# Autodesk Inventor assembly: C-SHA10_MIR_MIR_MIR1
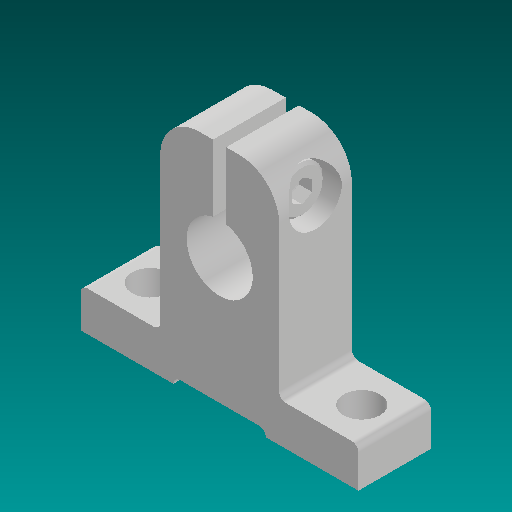
[picture p0: Inventor's stored thumbnail of the model, 512x512]
Saved by Autodesk Inventor 2020 (Build 240168000, 168)
## iProperties
Category: PARTsolutions
Company: MISUMI
Created: 2022-11-04
Part Number: C-SHA10_MIR_MIR_MIR1
Catalog Web Link: www.cadenas.de
Description: C-SHA-Economy Shaft Supports - T-Shaped/Slit
Vendor: MISUMI
Document SubType Name: Assembly
Designer: kanazawakotaro
Manufacturer: MISUMI
Mass: 6.70187 g
Surface Area: 40.5742 cm^2
Volume: 6.70187 cm^3
Density: 1 g/cm^3
Title: C-SHA10
Author: Cadenas PARTsolutions
Comments: Economy Shaft Supports - T-Shaped/Slit
PSOL_IDENT_0: {$CADENAS_DATA/23d-libs/misumi/metric/02_shaft_supports/c_sha_asmtab.prj},167 {VTYP=3D},{STYP=ASSTAB
PSOL_IDENT_1: },{NB=C-SHA10},{LINA=C-SHA10},{NN=C-SHA},{DATE=04.10.2022 06:54:20},{GEOMDATE=23.04.2021 02:50:35},{
PSOL_IDENT_2: VERSION=},{LINEID=10},{WBVAR=},{WBNUMERIC=}  {NB=C-SHA10},{LINA=C-SHA10},{KT=DUMMY},{PN=C-SHA10},{TY
PSOL_IDENT_3: PE=C-SHA},{D=10},{H=20},{H1=35},{T=11},{L1=32},{DD=5.5},{E=9.5},{S=6},{R=6},{L=42},{B=14},{W=18},{M=
PSOL_IDENT_4: M4},{R2=1},{W2=2.0},{M3D=4},{M3D2=6.0},{M3D3=8},{M3D4=4.3},{LB=10},{PPATH=c_sha/c_sha_asmtpl.prj}
NB: C-SHA10
NN: C-SHA
NT: Economy Shaft Supports - T-Shaped/Slit
NBSYN: $PN.
LINA: C-SHA10
CATALOG: Misumi
PN: C-SHA10
D: 10
H: 20
H1: 35
T: 11
L1: 32
DD: 5.5
E: 9.5
S: 6
R: 6
L: 42
B: 14
W: 18
M: M4
SUPPLIER: MISUMI
ARTICLENO: C-SHA10
BOMINFO: C-SHA10
CREATOR: CADENAS GmbH
## Documents named in this file (3)
- C:\Users\金澤航太郎\Documents\Inventor\kamuy2\Parts\C-SHA10_Autodesk_Inventor_2020_20221104\AIS2020\C-SHA10_MIR_MIR_MIR1.iam
- C:\Users\金澤航太郎\Documents\Inventor\kamuy2\Parts\C-SHA10_Autodesk_Inventor_2020_20221104\AIS2020\C-SHA10_b_MIR_MIR_MIR1.ipt
- C:\Users\金澤航太郎\Documents\Inventor\kamuy2\Parts\C-SHA10_Autodesk_Inventor_2020_20221104\AIS2020\BOLT4-10_MIR_MIR_MIR1.ipt
## Components (2 placed, 2 different names)
1. C-SHA10_b_MIR_MIR_MIR1:1 — to_bolt_Z@1 <-> to_cp_Z@2, to_bolt_XY@1 <-> to_cp_XY@2, to_bolt_YZ@1 <-> to_cp_YZ@2
2. BOLT4-10_MIR_MIR_MIR1:1 — to_bolt_Z@1 <-> to_cp_Z@2, to_bolt_XY@1 <-> to_cp_XY@2, to_bolt_YZ@1 <-> to_cp_YZ@2
## Relationships (3: Mate 2, Angle 1)
- to_bolt_Z@1 <-> to_cp_Z@2 [Mate]: C-SHA10_b_MIR_MIR_MIR1:1 ↔ BOLT4-10_MIR_MIR_MIR1:1
- to_bolt_XY@1 <-> to_cp_XY@2 [Mate]: C-SHA10_b_MIR_MIR_MIR1:1 ↔ BOLT4-10_MIR_MIR_MIR1:1
- to_bolt_YZ@1 <-> to_cp_YZ@2 [Angle] (0 deg): C-SHA10_b_MIR_MIR_MIR1:1 ↔ BOLT4-10_MIR_MIR_MIR1:1
